# Autodesk Inventor assembly: CougSat-1
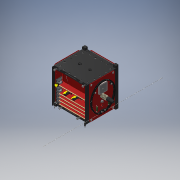
[picture p0: Inventor's stored thumbnail of the model, 180x180]
Saved by Autodesk Inventor 2018 (Build 220112000, 112)
## iProperties
Created: 2018-07-04
Part Number: CougSat-1
Document SubType Name: Assembly
Designer: Bradley
Mass: 728.063 g
Surface Area: 4946.19 cm^2
Volume: 325.846 cm^3
Density: 2.23438 g/cm^3
Author: Bradley
## Documents named in this file (12)
- D:\Users\Bradley\Documents\CougsInSpace\CougSat1-Hardware\CougSat1\CADModel\Native\CougSat-1.iam
- D:\Users\Bradley\Documents\CougsInSpace\CougSat1-Hardware\CougSat1-Structure\CADModel\Native\Structure.iam
- D:\Users\Bradley\Documents\CougsInSpace\CougSat1-Hardware\CougSat1-PowerBoard\CADModel\Native\EPS.iam
- D:\Users\Bradley\Documents\CougsInSpace\CougSat1-Hardware\CougSat1-PowerBoard\CADModel\Native\SolarPanelY.iam
- D:\Users\Bradley\Documents\CougsInSpace\CougSat1-Hardware\CougSat1-Backplane\CADModel\Native\Backplane.iam
- D:\Users\Bradley\Documents\CougsInSpace\CougSat1-Hardware\CougSat1-RadioBoard\CADModel\Native\RCS.iam
- D:\Users\Bradley\Documents\CougsInSpace\CougSat1-Hardware\CougSat1-Payload\CADModel\Native\Payload.iam
- D:\Users\Bradley\Documents\CougsInSpace\CougSat1-Hardware\CougSat1-Payload\CADModel\Native\PayloadGermination.iam
- D:\Users\Bradley\Documents\CougsInSpace\CougSat1-Hardware\CougSat1-AvionicBoard\CADModel\Native\Avionics.iam
- D:\Users\Bradley\Documents\CougsInSpace\CougSat1-Hardware\CougSat1-AvionicBoard\CADModel\Native\+XPanel.iam
- D:\Users\Bradley\Documents\CougsInSpace\CougSat1-Hardware\CougSat1-PowerBoard\CADModel\Native\SolarPanel+Z.iam
- D:\Users\Bradley\Documents\CougsInSpace\CougSat1-Hardware\CougSat1-PowerBoard\CADModel\Native\SolarPanel-X.iam
## Components (12 placed, 11 different names)
1. Structure:1 [sub-assembly] — Mate:1, Insert:1, Insert:2, Insert:3, Insert:4, Insert:5, Insert:6, Insert:7, Insert:8, Mate:2, Mate:3, Mate:4, Mate:5, Flush:3, Flush:4, Flush:5, Flush:6, Flush:7, Insert:11, Insert:12, Insert:13, Insert:14, Insert:15, Insert:16, Insert:17, Insert:18, Insert:19
2. EPS:1 [sub-assembly] — Flush:1, Mate:1, Flush:7
3. SolarPanelY:1 [sub-assembly] — Insert:1, Insert:2
4. SolarPanelY:2 [sub-assembly] — Insert:3, Insert:4
5. SolarPanel-X:1 [sub-assembly] — Insert:7, Insert:8
6. SolarPanel+Z:1 [sub-assembly] — Insert:5, Insert:6
7. Backplane:1 [sub-assembly] — Insert:13, Insert:14
8. RCS:1 [sub-assembly] — Mate:3, Flush:5, Flush:8
9. Payload:1 [sub-assembly] — Mate:2, Flush:6, Flush:9
10. PayloadGermination:1 [sub-assembly] — Mate:5, Flush:3, Flush:10, Insert:11, Insert:12
11. Avionics:1 [sub-assembly] — Mate:4, Flush:4, Flush:11
12. +XPanel:1 [sub-assembly] — Insert:15, Insert:16, Insert:17, Insert:18, Insert:19
## Relationships (32: Insert 17, Flush 10, Mate 5)
- Flush:1: EPS:1
- Mate:1 (0.04 mm): Structure:1 ↔ EPS:1
- Insert:1: Structure:1 ↔ SolarPanelY:1
- Insert:2: Structure:1 ↔ SolarPanelY:1
- Insert:3: Structure:1 ↔ SolarPanelY:2
- Insert:4: Structure:1 ↔ SolarPanelY:2
- Insert:5: Structure:1 ↔ SolarPanel+Z:1
- Insert:6: Structure:1 ↔ SolarPanel+Z:1
- Insert:7: Structure:1 ↔ SolarPanel-X:1
- Insert:8: Structure:1 ↔ SolarPanel-X:1
- Mate:2 (0.04 mm): Structure:1 ↔ Payload:1
- Mate:3 (0.04 mm): Structure:1 ↔ RCS:1
- Mate:4 (0.04 mm): Structure:1 ↔ Avionics:1
- Mate:5 (0.04 mm): Structure:1 ↔ PayloadGermination:1
- Flush:3 (1 mm): Structure:1 ↔ PayloadGermination:1
- Flush:4 (1 mm): Structure:1 ↔ Avionics:1
- Flush:5 (1 mm): Structure:1 ↔ RCS:1
- Flush:6 (1 mm): Structure:1 ↔ Payload:1
- Flush:7 (1 mm): Structure:1 ↔ EPS:1
- Flush:8: RCS:1
- Flush:9: Payload:1
- Flush:10: PayloadGermination:1
- Flush:11: Avionics:1
- Insert:11: Structure:1 ↔ PayloadGermination:1
- Insert:12: Structure:1 ↔ PayloadGermination:1
- Insert:13: Structure:1 ↔ Backplane:1
- Insert:14: Structure:1 ↔ Backplane:1
- Insert:15: Structure:1 ↔ +XPanel:1
- Insert:16: Structure:1 ↔ +XPanel:1
- Insert:17: Structure:1 ↔ +XPanel:1
- Insert:18: Structure:1 ↔ +XPanel:1
- Insert:19: Structure:1 ↔ +XPanel:1
